# Autodesk Inventor assembly: modul bund
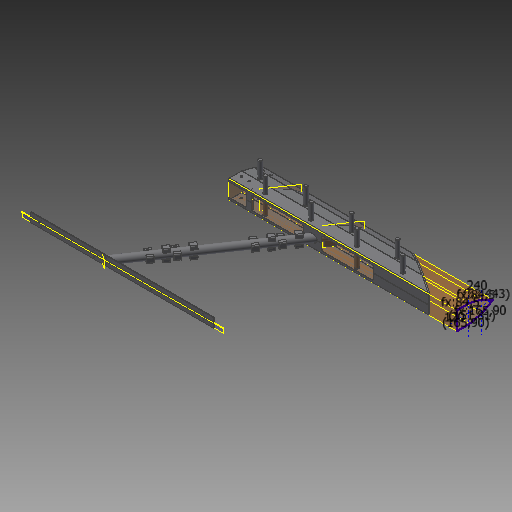
[picture p0: Inventor's stored thumbnail of the model, 512x512]
Saved by Autodesk Inventor 2018 (Build 220112000, 112)
## iProperties
Created: 2019-09-23
Part Number: modul bund
Document SubType Name: Assembly
Designer: loppen
Mass: 38633 g
Surface Area: 21634.5 cm^2
Volume: 4926.63 cm^3
Density: 7.84166 g/cm^3
Author: loppen
## Documents named in this file (18)
- Z:\trappe\modul bund.iam
- Z:\trappe\model.ipt
- Z:\trappe\vange bund.ipt
- Z:\trappe\bund vange-endeplade.ipt
- Z:\trappe\baluster\stilladssøjle.iam
- Z:\trappe\baluster-fod.ipt
- Z:\trappe\håndfang\håndfang bund.iam
- Z:\trappe\trappestift skrå.ipt
- Z:\trappe\trappestift.ipt
- Z:\trappe\skot.ipt
- Z:\trappe\skot opad.ipt
- Z:\trappe\modul\AIP\FEA\d09v3y4ww.fins
- Z:\trappe\modul\AIP\FEA\d09v3y4ww.fsat
- Z:\trappe\modul\AIP\FEA\d09v3y4ww.ftes
- Z:\trappe\modul\AIP\FEA\d09v3y4ww.fwiz
- Z:\trappe\modul\AIP\FEA\d09v3y50g.fmsh
- Z:\trappe\modul\AIP\FEA\d09v3y50h.fres
- Z:\trappe\trappe.xlsx
## Components (16 placed, 10 different names)
1. model:1 — Flush:1, Flush:2, Flush:3, Flush:4, Flush:5, Flush:6, Flush:7, Flush:8
2. vange bund:1 — Flush:1, Flush:2, Flush:3, Flush:4, Flush:5, Flush:6, Flush:7, Flush:8, Flush:9, Flush:10, Mate:2, Mate:3, Mate:4, Flush:11, Flush:12, Mate:6, Flush:13, Mate:10, Mate:11, Mate:12, Mate:13, Mate:14, Mate:15, Mate:16, Mate:17, Angle:1, Angle:2, Angle:3, Angle:4, Angle:5, Angle:6, Angle:7, Angle:8, Flush:14, Flush:15, Flush:16, Flush:17, Mate:18, Mate:19, Mate:20, Mate:21, Mate:22, Mate:23, Mate:24, Mate:25, Flush:19
3. bund vange-endeplade:1 — Flush:9, Flush:10, Mate:2, Mate:3
4. stilladssøjle:1 [sub-assembly] — Mate:4, Flush:11, Mate:5, Mate:7, Mate:8, Mate:9
5. baluster-fod:1 — Mate:5, Flush:12, Mate:6, Mate:7, Flush:18
6. håndfang bund:1 [sub-assembly] — Mate:8, Flush:13, Mate:9
7. trappestift skrå:1 — Mate:10, Angle:1, Mate:18
8. trappestift:1 — Mate:11, Angle:2, Flush:14
9. trappestift skrå:3 — Mate:12, Angle:3, Mate:19
10. trappestift:2 — Mate:13, Angle:4, Flush:15
11. trappestift skrå:5 — Mate:14, Angle:5, Mate:20
12. trappestift:3 — Mate:15, Angle:6, Flush:16
13. trappestift skrå:7 — Mate:16, Angle:7, Mate:21
14. trappestift:4 — Mate:17, Angle:8, Flush:17
15. skot:1 — Mate:22, Mate:23, Flush:18
16. skot opad:1 — Mate:24, Mate:25, Flush:19
## Relationships (51: Mate 24, Flush 19, Angle 8)
- Flush:1: model:1 ↔ vange bund:1
- Flush:2: model:1 ↔ vange bund:1
- Flush:3: model:1 ↔ vange bund:1
- Flush:4: model:1 ↔ vange bund:1
- Flush:5: model:1 ↔ vange bund:1
- Flush:6: model:1 ↔ vange bund:1
- Flush:7: model:1 ↔ vange bund:1
- Flush:8: model:1 ↔ vange bund:1
- Flush:9: vange bund:1 ↔ bund vange-endeplade:1
- Flush:10: vange bund:1 ↔ bund vange-endeplade:1
- Mate:2: vange bund:1 ↔ bund vange-endeplade:1
- Mate:3: vange bund:1 ↔ bund vange-endeplade:1
- Mate:4: vange bund:1 ↔ stilladssøjle:1
- Flush:11: vange bund:1 ↔ stilladssøjle:1
- Mate:5: stilladssøjle:1 ↔ baluster-fod:1
- Flush:12: vange bund:1 ↔ baluster-fod:1
- Mate:6 (43.655 mm): vange bund:1 ↔ baluster-fod:1
- Mate:7: stilladssøjle:1 ↔ baluster-fod:1
- Mate:8: stilladssøjle:1 ↔ håndfang bund:1
- Flush:13: vange bund:1 ↔ håndfang bund:1
- Mate:9 (-90 mm): stilladssøjle:1 ↔ håndfang bund:1
- Mate:10: vange bund:1 ↔ trappestift skrå:1
- Mate:11: vange bund:1 ↔ trappestift:1
- Mate:12: vange bund:1 ↔ trappestift skrå:3
- Mate:13: vange bund:1 ↔ trappestift:2
- Mate:14: vange bund:1 ↔ trappestift skrå:5
- Mate:15: vange bund:1 ↔ trappestift:3
- Mate:16: vange bund:1 ↔ trappestift skrå:7
- Mate:17: vange bund:1 ↔ trappestift:4
- Angle:1 (0 deg): vange bund:1 ↔ trappestift skrå:1
- Angle:2 (0 deg): vange bund:1 ↔ trappestift:1
- Angle:3 (0 deg): vange bund:1 ↔ trappestift skrå:3
- Angle:4 (0 deg): vange bund:1 ↔ trappestift:2
- Angle:5 (0 deg): vange bund:1 ↔ trappestift skrå:5
- Angle:6 (0 deg): vange bund:1 ↔ trappestift:3
- Angle:7 (0 deg): vange bund:1 ↔ trappestift skrå:7
- Angle:8 (0 deg): vange bund:1 ↔ trappestift:4
- Flush:14: vange bund:1 ↔ trappestift:1
- Flush:15: vange bund:1 ↔ trappestift:2
- Flush:16: vange bund:1 ↔ trappestift:3
- Flush:17: vange bund:1 ↔ trappestift:4
- Mate:18: vange bund:1 ↔ trappestift skrå:1
- Mate:19: vange bund:1 ↔ trappestift skrå:3
- Mate:20: vange bund:1 ↔ trappestift skrå:5
- Mate:21: vange bund:1 ↔ trappestift skrå:7
- Mate:22: vange bund:1 ↔ skot:1
- Mate:23 (1.659 mm): vange bund:1 ↔ skot:1
- Flush:18 (345.087 mm): baluster-fod:1 ↔ skot:1
- Mate:24 (2 mm): vange bund:1 ↔ skot opad:1
- Mate:25: vange bund:1 ↔ skot opad:1
- Flush:19 (13.5 mm): vange bund:1 ↔ skot opad:1
## Named parameters: sa_0 = 0, sa_1 = 0, sa_2 = -250000, trappestifter_dia = 25 mm, trappestifter_huldia = 25.8 mm, trappestifter_skraa_huldia = 26.6 mm, trappestifter_laengde = 228 mm, perforeringsbredde = 6 mm, perforeringshulprocent = 80 mm, perforeringshullaengde = 62.8 mm, perforeringshullaengde_top = 61 mm, perforeringshullaengde_bund = 61.6 mm, perforeringsoffset = 8 mm, perforeringsoffset_top = 8 mm, perforeringsoffset_bund = 8 mm, laskehul_dia = 13 mm, haandfang_offset_fra_top = 90 mm, trappevinkel = 34.3 deg, balusterhul_udvidelse = 1 mm, pladetykkelse = 3 mm
note: some values were not read from the file. Shown as the stored number, unit unknown: "sa_0", "sa_1", "sa_2".
